# Autodesk Inventor assembly: FR-01assembled
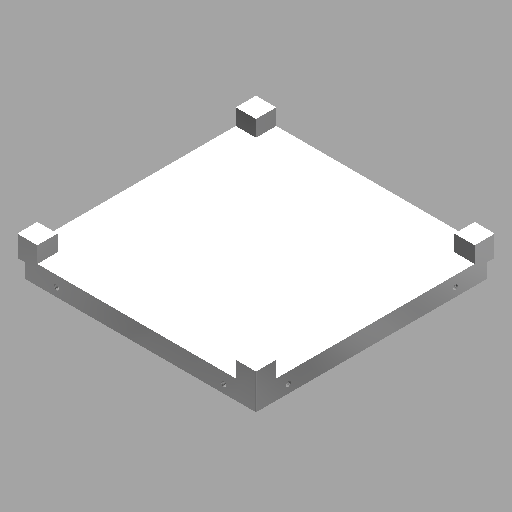
[picture p0: Inventor's stored thumbnail of the model, 512x512]
Saved by Autodesk Inventor 2022 (Build 260153000, 153)
## iProperties
Created: 2021-10-08
Part Number: FR-01assembled
Document SubType Name: Assembly
Designer: Bowen O'Steen
Author: Bowen O'Steen
## Documents named in this file (2)
- C:\Users\gwhen\OneDrive\Desktop\Vault\Designs\MEMESat\MemeSat\Engineering Data\MemeSat\Assembly\FR-01assembled.iam
- C:\Users\gwhen\OneDrive\Desktop\Vault\Designs\MEMESat\MemeSat\Engineering Data\MemeSat\Frame\FR-01.ipt
## Components (1 placed, 1 different names)
1. FR-01:1 — Mate:1, Mate:2, Flush:1
## Relationships (3: Mate 2, Flush 1)
- Mate:1: FR-01:1
- Mate:2: FR-01:1
- Flush:1: FR-01:1
